# Autodesk Inventor assembly: Zespół1
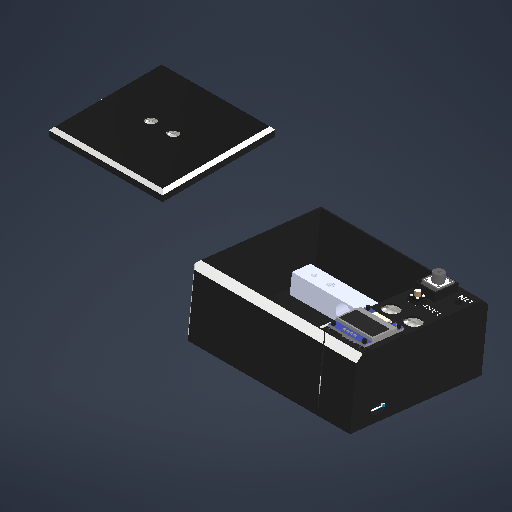
[picture p0: Inventor's stored thumbnail of the model, 512x512]
Saved by Autodesk Inventor 2026.2 (Build 302298010, 298A)
## iProperties
Created: 2026-03-26
Part Number: Zespół1
Document SubType Name: Assembly
Designer: User
Author: User
## Documents named in this file (11)
- C:\Users\testo\Documents\Scale\Hardware\Model\Zespół1.iam
- C:\Users\testo\Documents\Scale\Hardware\Model\taca.ipt
- C:\Users\testo\Documents\Scale\Hardware\Model\bridz.ipt
- C:\Users\testo\Documents\Scale\Hardware\Model\klappa.ipt
- C:\Users\testo\Documents\Scale\Hardware\Model\TP4056_Charging_Module_Type_C\TP4056_Charging_Module_Type_C\TP4056_Charging_Module_Type_C.ipt
- C:\Users\testo\Documents\Scale\Hardware\Model\GUZIK.ipt
- C:\Users\testo\Documents\Scale\Hardware\Model\92000A328_Passivated 18-8 Stainless Steel Pan Head Phillips Screws\92000A328_Passivated 18-8 Stainless Steel Pan Head Phillips Screws\92000A328_Passivated 18-8 Stainle.ipt
- C:\Users\testo\Documents\Scale\Hardware\Model\92000A220_Passivated 18-8 Stainless Steel Pan Head Phillips Screws\92000A220_Passivated 18-8 Stainless Steel Pan Head Phillips Screws\92000A220_Passivated 18-8 Stainle.ipt
- C:\Users\testo\Documents\Scale\Hardware\Model\mypushbutton\mypushbutton\mypushbutton.ipt
- C:\Users\testo\Documents\Inventor\0.9 inch I2C OLED 128×64 Display Module_jhalak\0.9 inch I2C OLED 128×64 Display Module_jhalak.ipt
- C:\Users\testo\Documents\Inventor\loadcell_10kg_tal220B\loadcell_10kg_tal220B.ipt
## Components (12 placed, 10 different names)
1. taca:1 — Obrotowe:8
2. bridz:1 — Sztywne:1, Sztywne:2, Równoległe:1, Zestawiające:1, Równoległe:2
3. klappa:1 — Sztywne:1, Obrotowe:6, Obrotowe:7, Sztywne:4, Obrotowe:9, Obrotowe:10
4. TP4056_Charging_Module_Type_C:1 — Sztywne:2
5. GUZIK:1 — Obrotowe:6
6. mypushbutton:1 — Sztywne:4
7. 0.9 inch I2C OLED 128×64 Display Module_jhalak:2 — Obrotowe:9, Obrotowe:10
8. loadcell_10kg_tal220B:2 — Równoległe:1, Zestawiające:1, Równoległe:2
9. 92000A328_Passivated 18-8 Stainle:1 — Obrotowe:7
10. 92000A328_Passivated 18-8 Stainle:2
11. 92000A220_Passivated 18-8 Stainle:1 — Obrotowe:8
12. 92000A220_Passivated 18-8 Stainle:2
## Component patterns: (2 elements, first: 92000A328_Passivated 18-8 Stainle:1), (2 elements, first: 92000A220_Passivated 18-8 Stainle:1)
## Relationships (11: RevoluteJoint 5, WeldJoint 3, Flush 2, Mate 1)
- Sztywne:1 [WeldJoint] (12.7 mm): bridz:1 ↔ klappa:1
- Sztywne:2 [WeldJoint] (0.4 mm): bridz:1 ↔ TP4056_Charging_Module_Type_C:1
- Obrotowe:6 [RevoluteJoint] (-2 mm): klappa:1 ↔ GUZIK:1
- Obrotowe:7 [RevoluteJoint] (-21 mm): klappa:1 ↔ 92000A328_Passivated 18-8 Stainle:1
- Obrotowe:8 [RevoluteJoint] (-10 mm): taca:1 ↔ 92000A220_Passivated 18-8 Stainle:1
- Sztywne:4 [WeldJoint]: klappa:1 ↔ mypushbutton:1
- Obrotowe:9 [RevoluteJoint]: klappa:1 ↔ 0.9 inch I2C OLED 128×64 Display Module_jhalak:2
- Obrotowe:10 [RevoluteJoint]: klappa:1 ↔ 0.9 inch I2C OLED 128×64 Display Module_jhalak:2
- Równoległe:1 [Flush]: bridz:1 ↔ loadcell_10kg_tal220B:2
- Zestawiające:1 [Mate]: bridz:1 ↔ loadcell_10kg_tal220B:2
- Równoległe:2 [Flush]: bridz:1 ↔ loadcell_10kg_tal220B:2
